# Autodesk Inventor assembly: body
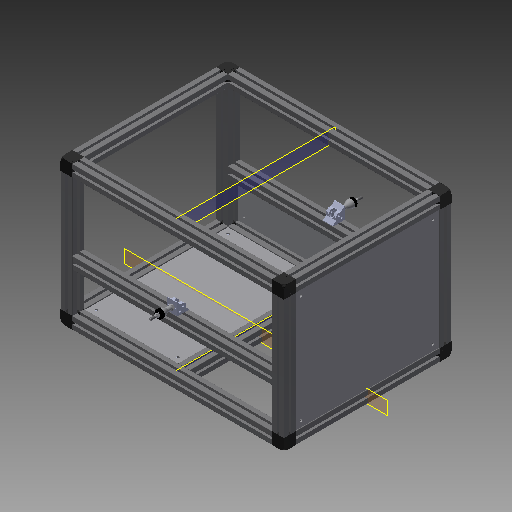
[picture p0: Inventor's stored thumbnail of the model, 512x512]
Saved by Autodesk Inventor 2021.3 (Build 253353000, 353)
## iProperties
Created: 2021-07-09
Part Number: body
Material: 一般
Document SubType Name: Assembly
Designer: gisen
Mass: 47360.5 g
Surface Area: 66475.9 cm^2
Volume: 35407.1 cm^3
Density: 1.3376 g/cm^3
Author: gisen
## Documents named in this file (11)
- C:\Users\gisen\workspace\beetle_inventor_model\body\body.iam
- C:\Users\gisen\workspace\beetle_inventor_model\body\AFS-3030-360.ipt
- C:\Users\gisen\workspace\beetle_inventor_model\body\AFS-3030-300.ipt
- C:\Users\gisen\workspace\beetle_inventor_model\suspension\RBID6\RBID6.iam
- C:\Users\gisen\workspace\beetle_inventor_model\suspension\frame\ABLB-3025-6.ipt
- C:\Users\gisen\workspace\beetle_inventor_model\body\AFS-3030-500.ipt
- C:\Users\gisen\workspace\beetle_inventor_model\body\ABC-3030-6.ipt
- C:\Users\gisen\workspace\beetle_inventor_model\body\ABLD-30-6-N-T.ipt
- C:\Users\gisen\workspace\beetle_inventor_model\body\panel\bottom_panel.ipt
- C:\Users\gisen\workspace\beetle_inventor_model\body\panel\front_panel.ipt
- C:\Users\gisen\workspace\beetle_inventor_model\body\panel\side_panel.ipt
## Components (34 placed, 10 different names)
1. AFS-3030-500:1 — フラッシュ:1, メイト:1, メイト:2, メイト:3, メイト:46, メイト:10, フラッシュ:5, 対称度:1, メイト:14, フラッシュ:15, メイト:33, メイト:45, メイト:66, メイト:67, メイト:75, メイト:84
2. AFS-3030-360:1 — フラッシュ:1, メイト:1, メイト:2, メイト:4, メイト:9, 対称度:2, メイト:12, メイト:65, メイト:71, メイト:73, メイト:74
3. AFS-3030-300:1 — メイト:3, メイト:4, メイト:46, フラッシュ:4, フラッシュ:7, メイト:53, メイト:62, メイト:83
4. AFS-3030-500:2 — メイト:9, 角度:1, 対称度:1, メイト:11, フラッシュ:17, フラッシュ:19, メイト:70, メイト:72, メイト:76, メイト:79
5. AFS-3030-360:2 — メイト:10, フラッシュ:5, 対称度:2, メイト:13
6. AFS-3030-300:2 — フラッシュ:4, メイト:44, メイト:52, メイト:61, メイト:81
7. AFS-3030-300:3 — フラッシュ:6, メイト:13, メイト:14, メイト:32, メイト:54, メイト:55, メイト:60
8. AFS-3030-300:4 — フラッシュ:6, メイト:11, フラッシュ:7, メイト:12, メイト:27, メイト:28, メイト:47, メイト:51, メイト:63, メイト:64
9. AFS-3030-500:4
10. AFS-3030-360:3 — メイト:27, 対称度:3
11. AFS-3030-500:5 — メイト:28, メイト:47
12. AFS-3030-360:4 — 対称度:3, メイト:82, フラッシュ:21
13. AFS-3030-500:6 — フラッシュ:15, メイト:32, メイト:33, メイト:36, メイト:39, フラッシュ:18, フラッシュ:22
14. RBID6:1 [sub-assembly] — メイト:34, メイト:35
15. ABLB-3025-6:1 — メイト:34, メイト:35, メイト:36, メイト:38, メイト:39
16. AFS-3030-500:7 — フラッシュ:17, メイト:44, フラッシュ:18
17. RBID6:2 [sub-assembly]
18. ABLB-3025-6:2 — フラッシュ:16
19. AFS-3030-360:5 — フラッシュ:19, メイト:45, フラッシュ:20, メイト:68, メイト:69, メイト:78
20. ABC-3030-6:1 — メイト:48, メイト:53, メイト:49
21. ABC-3030-6:2 — メイト:48, メイト:51
22. ABC-3030-6:3 — メイト:49, メイト:50, メイト:54, メイト:55
23. ABC-3030-6:4 — メイト:50, メイト:52
24. ABC-3030-6:5 — メイト:61
25. ABC-3030-6:6 — メイト:59, メイト:63, メイト:64
26. ABC-3030-6:7 — メイト:60
27. ABC-3030-6:8 — メイト:59, メイト:62
28. ABLD-30-6-N-T:1 — メイト:65, メイト:66, メイト:74
29. ABLD-30-6-N-T:2 — メイト:71, メイト:72, メイト:73, メイト:80
30. ABLD-30-6-N-T:3 — メイト:69, メイト:70, メイト:76
31. ABLD-30-6-N-T:4 — メイト:67, メイト:68, メイト:75
32. bottom_panel:1 — メイト:78, メイト:79, メイト:80
33. front_panel:1 — メイト:81, メイト:82, フラッシュ:21
34. side_panel:1 — メイト:83, メイト:84, フラッシュ:22
## Relationships (95: Mate 74, Flush 17, Symmetry 3, Angle 1)
- フラッシュ:1 [Flush]: AFS-3030-500:1 ↔ AFS-3030-360:1
- メイト:1 [Mate]: AFS-3030-500:1 ↔ AFS-3030-360:1
- メイト:2 [Mate]: AFS-3030-500:1 ↔ AFS-3030-360:1
- メイト:3 [Mate]: AFS-3030-500:1 ↔ AFS-3030-300:1
- メイト:4 [Mate]: AFS-3030-360:1 ↔ AFS-3030-300:1
- メイト:46 [Mate]: AFS-3030-500:1 ↔ AFS-3030-300:1
- [Flush]: AFS-3030-500:2 ↔ AFS-3030-360:2
- [Mate]: AFS-3030-500:2 ↔ AFS-3030-360:2
- [Mate]: AFS-3030-500:2 ↔ AFS-3030-360:2
- [Mate]: AFS-3030-500:2 ↔ AFS-3030-300:2
- [Mate]: AFS-3030-360:2 ↔ AFS-3030-300:2
- フラッシュ:4 [Flush]: AFS-3030-300:1 ↔ AFS-3030-300:2
- メイト:9 [Mate]: AFS-3030-360:1 ↔ AFS-3030-500:2
- メイト:10 [Mate]: AFS-3030-500:1 ↔ AFS-3030-360:2
- フラッシュ:5 [Flush]: AFS-3030-500:1 ↔ AFS-3030-360:2
- 角度:1 [Angle] (0 deg): AFS-3030-500:2
- メイト:37 [Mate]
- 対称度:1 [Symmetry]: AFS-3030-500:1 ↔ AFS-3030-500:2
- 対称度:2 [Symmetry]: AFS-3030-360:1 ↔ AFS-3030-360:2
- フラッシュ:6 [Flush]: AFS-3030-300:3 ↔ AFS-3030-300:4
- メイト:11 [Mate]: AFS-3030-500:2 ↔ AFS-3030-300:4
- フラッシュ:7 [Flush]: AFS-3030-300:1 ↔ AFS-3030-300:4
- メイト:12 [Mate]: AFS-3030-360:1 ↔ AFS-3030-300:4
- メイト:13 [Mate]: AFS-3030-360:2 ↔ AFS-3030-300:3
- メイト:14 [Mate]: AFS-3030-500:1 ↔ AFS-3030-300:3
- [Flush]: AFS-3030-500:4 ↔ AFS-3030-360:3
- [Mate]: AFS-3030-500:4 ↔ AFS-3030-360:3
- [Mate]: AFS-3030-500:4 ↔ AFS-3030-360:3
- [Flush]: AFS-3030-500:5 ↔ AFS-3030-360:4
- [Mate]: AFS-3030-500:5 ↔ AFS-3030-360:4
- [Mate]: AFS-3030-500:5 ↔ AFS-3030-360:4
- [Mate]: AFS-3030-360:3 ↔ AFS-3030-500:5
- [Mate]: AFS-3030-500:4 ↔ AFS-3030-360:4
- [Flush]: AFS-3030-500:4 ↔ AFS-3030-360:4
- メイト:27 [Mate]: AFS-3030-300:4 ↔ AFS-3030-360:3
- メイト:28 [Mate]: AFS-3030-300:4 ↔ AFS-3030-500:5
- メイト:47 [Mate]: AFS-3030-300:4 ↔ AFS-3030-500:5
- フラッシュ:15 [Flush]: AFS-3030-500:1 ↔ AFS-3030-500:6
- メイト:32 [Mate]: AFS-3030-300:3 ↔ AFS-3030-500:6
- メイト:33 [Mate] (100 mm): AFS-3030-500:1 ↔ AFS-3030-500:6
- メイト:34 [Mate]: RBID6:1 ↔ ABLB-3025-6:1
- メイト:35 [Mate]: RBID6:1 ↔ ABLB-3025-6:1
- メイト:36 [Mate]: AFS-3030-500:6 ↔ ABLB-3025-6:1
- 対称度:3 [Symmetry]: AFS-3030-360:3 ↔ AFS-3030-360:4
- メイト:38 [Mate]: ABLB-3025-6:1
- メイト:39 [Mate] (-15 mm): AFS-3030-500:6 ↔ ABLB-3025-6:1
- [Mate]: RBID6:2 ↔ ABLB-3025-6:2
- [Mate]: RBID6:2 ↔ ABLB-3025-6:2
- [Mate]: AFS-3030-500:7 ↔ ABLB-3025-6:2
- [Mate] (-15 mm): AFS-3030-500:7 ↔ ABLB-3025-6:2
- フラッシュ:16 [Flush]: ABLB-3025-6:2
- フラッシュ:17 [Flush]: AFS-3030-500:2 ↔ AFS-3030-500:7
- メイト:44 [Mate]: AFS-3030-300:2 ↔ AFS-3030-500:7
- フラッシュ:18 [Flush]: AFS-3030-500:6 ↔ AFS-3030-500:7
- フラッシュ:19 [Flush]: AFS-3030-500:2 ↔ AFS-3030-360:5
- メイト:45 [Mate]: AFS-3030-500:1 ↔ AFS-3030-360:5
- フラッシュ:20 [Flush]: AFS-3030-360:5
- メイト:48 [Mate]: ABC-3030-6:1 ↔ ABC-3030-6:2
- メイト:49 [Mate]: ABC-3030-6:1 ↔ ABC-3030-6:3
- メイト:50 [Mate]: ABC-3030-6:3 ↔ ABC-3030-6:4
- メイト:51 [Mate]: AFS-3030-300:4 ↔ ABC-3030-6:2
- メイト:52 [Mate]: AFS-3030-300:2 ↔ ABC-3030-6:4
- メイト:53 [Mate]: AFS-3030-300:1 ↔ ABC-3030-6:1
- メイト:54 [Mate]: AFS-3030-300:3 ↔ ABC-3030-6:3
- メイト:55 [Mate]: AFS-3030-300:3 ↔ ABC-3030-6:3
- [Mate]: ABC-3030-6:5 ↔ ABC-3030-6:6
- [Mate]: ABC-3030-6:5 ↔ ABC-3030-6:7
- [Mate]: ABC-3030-6:7 ↔ ABC-3030-6:8
- メイト:59 [Mate]: ABC-3030-6:6 ↔ ABC-3030-6:8
- メイト:60 [Mate]: AFS-3030-300:3 ↔ ABC-3030-6:7
- メイト:61 [Mate]: AFS-3030-300:2 ↔ ABC-3030-6:5
- メイト:62 [Mate]: AFS-3030-300:1 ↔ ABC-3030-6:8
- メイト:63 [Mate]: AFS-3030-300:4 ↔ ABC-3030-6:6
- メイト:64 [Mate]: AFS-3030-300:4 ↔ ABC-3030-6:6
- メイト:65 [Mate]: AFS-3030-360:1 ↔ ABLD-30-6-N-T:1
- メイト:66 [Mate]: AFS-3030-500:1 ↔ ABLD-30-6-N-T:1
- メイト:67 [Mate]: AFS-3030-500:1 ↔ ABLD-30-6-N-T:4
- メイト:68 [Mate]: AFS-3030-360:5 ↔ ABLD-30-6-N-T:4
- メイト:69 [Mate]: AFS-3030-360:5 ↔ ABLD-30-6-N-T:3
- メイト:70 [Mate]: AFS-3030-500:2 ↔ ABLD-30-6-N-T:3
- メイト:71 [Mate]: AFS-3030-360:1 ↔ ABLD-30-6-N-T:2
- メイト:72 [Mate]: AFS-3030-500:2 ↔ ABLD-30-6-N-T:2
- メイト:73 [Mate] (-15 mm): AFS-3030-360:1 ↔ ABLD-30-6-N-T:2
- メイト:74 [Mate] (-15 mm): AFS-3030-360:1 ↔ ABLD-30-6-N-T:1
- メイト:75 [Mate] (-15 mm): AFS-3030-500:1 ↔ ABLD-30-6-N-T:4
- メイト:76 [Mate] (-15 mm): AFS-3030-500:2 ↔ ABLD-30-6-N-T:3
- メイト:78 [Mate]: AFS-3030-360:5 ↔ bottom_panel:1
- メイト:79 [Mate]: AFS-3030-500:2 ↔ bottom_panel:1
- メイト:80 [Mate]: ABLD-30-6-N-T:2 ↔ bottom_panel:1
- メイト:81 [Mate]: AFS-3030-300:2 ↔ front_panel:1
- メイト:82 [Mate]: AFS-3030-360:4 ↔ front_panel:1
- フラッシュ:21 [Flush] (2 mm): AFS-3030-360:4 ↔ front_panel:1
- メイト:83 [Mate]: AFS-3030-300:1 ↔ side_panel:1
- メイト:84 [Mate]: AFS-3030-500:1 ↔ side_panel:1
- フラッシュ:22 [Flush] (2 mm): AFS-3030-500:6 ↔ side_panel:1
## Named parameters: d1489_d1485 = 0 mm, d1490_d1486 = 0 mm, d1491_d1487 = 0 mm, d1492_d1488 = 0 mm, d1493_d1483 = 0 mm, d1494_d1484 = 0 mm, d1515_d1485 = 0 mm, d1516_d1489_d1485 = 0 mm, d1517_d1493_d1483 = 0 mm, d1518_d1494_d1484 = 0 mm, d1519_d1495 = 0 mm, d1520_d1496 = 0 mm, d1521_d1497 = 0 mm, d1522_d1483 = 0 mm, d1523_d1484 = 0 mm, d1542_d1541 = -15 mm, d1543_d1536 = 0 mm, d1544_d1537 = 0 mm, d1545_d1538 = 0 mm, d1561_d1553 = 0 mm, d1562_d1554 = 0 mm, d1563_d1555 = 0 mm
